# Autodesk Inventor assembly: skellett
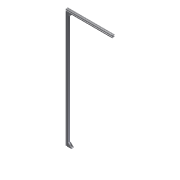
[picture p0: Inventor's stored thumbnail of the model, 180x180]
Saved by Autodesk Inventor 2014 SP1 (Build 180222100, 222)
## iProperties
Created: 2015-02-04
Part Number: skellett
Document SubType Name: Assembly
Designer: Simen
Author: Simen
## Documents named in this file (6)
- C:\Users\Simen\Documents\git\Eit\skjellet\skellett.iam
- C:\Users\Simen\Documents\git\Eit\skjellet\KHFS5_2020_1000.ipt
- C:\Users\Simen\Documents\git\Eit\skjellet\KHFS5_2020_400.ipt
- C:\Users\Simen\Documents\git\Eit\skjellet\HBLFSL5hblfsn5.ipt
- C:\Users\Simen\Documents\git\Eit\skjellet\HBLFSN5.iam
- C:\Users\Simen\Documents\git\Eit\skjellet\mutterOgSkrue.iam
## Components (5 placed, 5 different names)
1. KHFS5-2020-400:1 — Flush:3, Mate:2, Flush:4
2. KHFS5-2020-1000:1 — Mate:1, Flush:1, Flush:2, Flush:3, Flush:4
3. HBLFSN5:1 [sub-assembly]
4. HBLFSL5hblfsn5:1 — Mate:1, Flush:1, Flush:2, Mate:2
5. mutterOgSkrue:1 [sub-assembly]
## Relationships (12: Mate 6, Flush 6)
- Mate:1: KHFS5-2020-1000:1 ↔ HBLFSL5hblfsn5:1
- Flush:1: KHFS5-2020-1000:1 ↔ HBLFSL5hblfsn5:1
- Flush:2 (3 mm): KHFS5-2020-1000:1 ↔ HBLFSL5hblfsn5:1
- Flush:3: KHFS5-2020-400:1 ↔ KHFS5-2020-1000:1
- Mate:2: KHFS5-2020-400:1 ↔ HBLFSL5hblfsn5:1
- Flush:4: KHFS5-2020-400:1 ↔ KHFS5-2020-1000:1
- [Mate]: KHFS5-2020-1000:1 ↔ HBLFSN5:1
- [Flush]: KHFS5-2020-1000:1 ↔ HBLFSN5:1
- [Flush]: KHFS5-2020-1000:1 ↔ HBLFSN5:1
- [Mate]: KHFS5-2020-1000:1 ↔ mutterOgSkrue:1
- [Mate]: KHFS5-2020-1000:1 ↔ mutterOgSkrue:1
- [Mate]: HBLFSN5:1 ↔ mutterOgSkrue:1
## Named parameters: d8_d2 = 0 mm, d9_d0 = 0 mm, d11_d5 = 0 mm
